# Autodesk Inventor assembly: REAR B Battery Pack - Alt
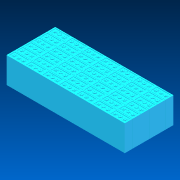
[picture p0: Inventor's stored thumbnail of the model, 180x180]
Saved by Autodesk Inventor 2012 (Build 160160000, 160)
## iProperties
Created: 2012-07-04
Part Number: REAR B Battery Pack - Alt
Document SubType Name: Assembly
Designer: Hemant
Author: Hemant
## Documents named in this file (2)
- C:\Users\Hemant\Documents\Battery Boxes\Batteries\REAR B Battery Pack - Alt.iam
- C:\Users\Hemant\Documents\Battery Boxes\Batteries\CALB100AH final.ipt
## Components (42 placed, 1 different names)
1. CALB100AH final:1
2. CALB100AH final:2
3. CALB100AH final:3
4. CALB100AH final:4
5. CALB100AH final:5
6. CALB100AH final:6
7. CALB100AH final:7
8. CALB100AH final:8
9. CALB100AH final:9
10. CALB100AH final:10
11. CALB100AH final:11
12. CALB100AH final:12
13. CALB100AH final:13
14. CALB100AH final:14
15. CALB100AH final:15
16. CALB100AH final:16
17. CALB100AH final:17
18. CALB100AH final:18
19. CALB100AH final:19
20. CALB100AH final:20
21. CALB100AH final:21
22. CALB100AH final:22
23. CALB100AH final:23
24. CALB100AH final:24
25. CALB100AH final:25
26. CALB100AH final:26
27. CALB100AH final:27
28. CALB100AH final:28
29. CALB100AH final:29
30. CALB100AH final:30
31. CALB100AH final:31
32. CALB100AH final:32
33. CALB100AH final:33
34. CALB100AH final:34
35. CALB100AH final:35
36. CALB100AH final:36
37. CALB100AH final:37
38. CALB100AH final:38
39. CALB100AH final:39
40. CALB100AH final:40
41. CALB100AH final:41
42. CALB100AH final:42
## Component patterns: (42 elements, first: CALB100AH final:1)
